# Autodesk Inventor assembly: LeftShoulderCrankUnit
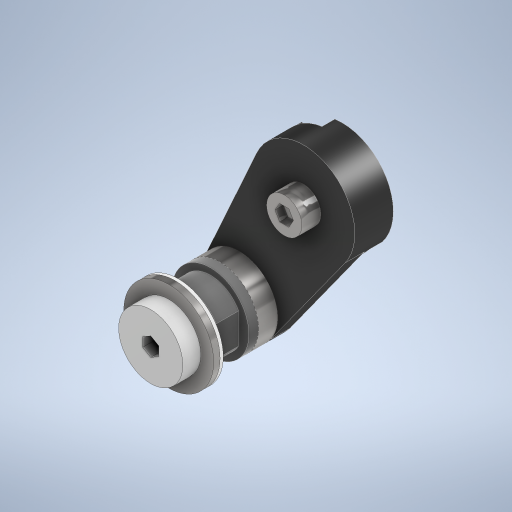
[picture p0: Inventor's stored thumbnail of the model, 512x512]
Saved by Autodesk Inventor 2024.2 (Build 282272000, 272)
## iProperties
Created: 2024-01-06
Part Number: LeftShoulderCrankUnit
Document SubType Name: Assembly
Designer: Masato Kubotera
Author: Masato Kubotera
## Documents named in this file (8)
- C:\Users\masato\OneDrive - Chiba Institute of Technology\CIT Brains\RoboCup2024\Mechanic\SUSTAINA-OP2\NativeFiles\Boby\UpperLimb\Shoulders\LeftShoulderCrankUnit.iam
- C:\Users\masato\OneDrive - Chiba Institute of Technology\CIT Brains\RoboCup2024\Mechanic\SUSTAINA-OP2\NativeFiles\Boby\COTS\Washers\Metal\UUW-0412-30H.ipt
- C:\Users\masato\OneDrive - Chiba Institute of Technology\CIT Brains\RoboCup2024\Mechanic\SUSTAINA-OP2\NativeFiles\Boby\COTS\Bushes\LED-0606.ipt
- C:\Users\masato\OneDrive - Chiba Institute of Technology\CIT Brains\RoboCup2024\Mechanic\SUSTAINA-OP2\NativeFiles\Boby\COTS\Screws\ScrewsWithShoulder\DBSY4-8-6.ipt
- C:\Users\masato\OneDrive - Chiba Institute of Technology\CIT Brains\RoboCup2024\Mechanic\SUSTAINA-OP2\NativeFiles\Boby\CommonDesignedComponents\SlashCutLongCrankFrame.ipt
- C:\Users\masato\OneDrive - Chiba Institute of Technology\CIT Brains\RoboCup2024\Mechanic\SUSTAINA-OP2\NativeFiles\Boby\COTS\Washers\Metal\UUW-0614-10H.ipt
- C:\Users\masato\OneDrive - Chiba Institute of Technology\CIT Brains\RoboCup2024\Mechanic\SUSTAINA-OP2\NativeFiles\Boby\COTS\Washers\Resin\TT-0614-05.ipt
- C:\Users\masato\OneDrive - Chiba Institute of Technology\CIT Brains\RoboCup2024\Mechanic\SUSTAINA-OP2\NativeFiles\Boby\COTS\Screws\CapScrew\UC-0308.ipt
## Components (7 placed, 7 different names)
1. SlashCutLongCrankFrame:1 — Angle:1, Mate:1, Mate:2, Insert:1, Insert:3
2. LED-0606:1 — Insert:2, Angle:2
3. UC-0308:1 — Insert:3
4. UUW-0614-10H:1 — Insert:4, Insert:5
5. TT-0614-05:1 — Insert:4
6. UUW-0412-30H:1 — Insert:1, Insert:2, Insert:6
7. DBSY4-8-6:1 — Insert:5, Insert:6
## Relationships (10: Insert 6, Angle 2, Mate 2)
- Angle:1 (30 deg): SlashCutLongCrankFrame:1
- Angle:2 (0 deg): LED-0606:1
- Mate:1: SlashCutLongCrankFrame:1
- Mate:2 (21.25 mm): SlashCutLongCrankFrame:1
- Insert:1: SlashCutLongCrankFrame:1 ↔ UUW-0412-30H:1
- Insert:2: LED-0606:1 ↔ UUW-0412-30H:1
- Insert:3: SlashCutLongCrankFrame:1 ↔ UC-0308:1
- Insert:4: UUW-0614-10H:1 ↔ TT-0614-05:1
- Insert:5: UUW-0614-10H:1 ↔ DBSY4-8-6:1
- Insert:6: UUW-0412-30H:1 ↔ DBSY4-8-6:1
